# Autodesk Inventor assembly: Podstawa_zlozona+Sruby
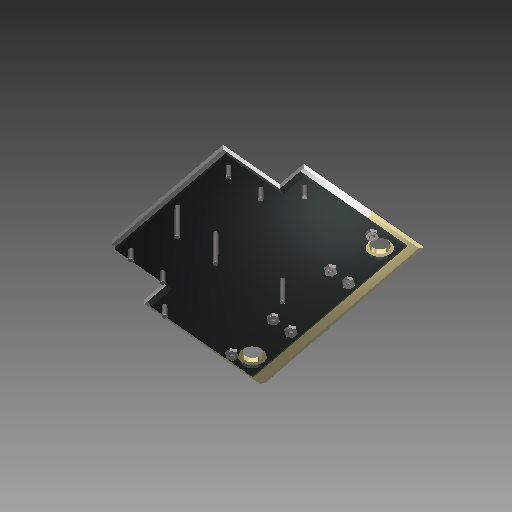
[picture p0: Inventor's stored thumbnail of the model, 512x512]
Saved by Autodesk Inventor 2017 (Build 210142000, 142)
## iProperties
Created: 2016-11-21
Part Number: Podstawa_zlozona+Sruby
Document SubType Name: Assembly
Designer: Shichi
Author: Shichi
## Documents named in this file (7)
- C:\Users\Shichi\Desktop\TooStronk\Podstawy\Podstawa_zlozona+Sruby.iam
- C:\Users\Shichi\Desktop\TooStronk\Podstawy\Podstawa_zlozona.iam
- C:\Users\Shichi\Documents\Inventor\Content Center Files\R2017\en-US\AS 1110\AS 1110 - M2,5 x 12.ipt
- C:\Users\Shichi\Documents\Inventor\Content Center Files\R2017\en-US\AS 1112 (2)\AS 1112 - M2,5  Type 5.ipt
- C:\Users\Shichi\Documents\Inventor\Content Center Files\R2017\en-US\AS 1110\AS 1110 - M2,5 x 8.ipt
- C:\Users\Shichi\Documents\Inventor\Content Center Files\R2017\en-US\AS 1110\AS 1110 - M2,5 x 20.ipt
- C:\Users\Shichi\Documents\Inventor\Content Center Files\R2017\en-US\AS 1110\AS 1110 - M2,5 x 25.ipt
## Components (22 placed, 6 different names)
1. Podstawa_zlozona:1 [sub-assembly] — Insert:1, Insert:2, Insert:4, Insert:5, Insert:6, Insert:7, Insert:10, Insert:11, Insert:12, Insert:13, Insert:14, Insert:15, Insert:16, Insert:17, Insert:18, Insert:19, Insert:20, Insert:21, Insert:22, Insert:23, Insert:24
2. AS 1110 - Metric M2,5 x 12:1 — Insert:4
3. AS 1110 - Metric M2,5 x 8:1 — Insert:11
4. AS 1110 - Metric M2,5 x 12:2 — Insert:2
5. AS 1110 - Metric M2,5 x 12:3 — Insert:5
6. AS 1110 - Metric M2,5 x 12:5 — Insert:1
7. AS 1110 - Metric M2,5 x 12:6 — Insert:6
8. AS 1110 - Metric M2,5 x 8:3 — Insert:15
9. AS 1110 - Metric M2,5 x 8:4 — Insert:14
10. AS 1110 - Metric M2,5 x 8:5 — Insert:13
11. AS 1110 - Metric M2,5 x 8:6 — Insert:12
12. AS 1110 - Metric M2,5 x 8:7 — Insert:10
13. AS 1112 (2) - Metric M2,5  Type 5:3 — Insert:20
14. AS 1112 (2) - Metric M2,5  Type 5:4 — Insert:21
15. AS 1112 (2) - Metric M2,5  Type 5:8 — Insert:17
16. AS 1112 (2) - Metric M2,5  Type 5:9 — Insert:18
17. AS 1112 (2) - Metric M2,5  Type 5:10 — Insert:19
18. AS 1112 (2) - Metric M2,5  Type 5:11 — Insert:16
19. AS 1110 - Metric M2,5 x 12:7 — Insert:7
20. AS 1110 - Metric M2,5 x 20:1 — Insert:22
21. AS 1110 - Metric M2,5 x 25:1 — Insert:24
22. AS 1110 - Metric M2,5 x 25:2 — Insert:23
## Relationships (21: Insert 21)
- Insert:1: Podstawa_zlozona:1 ↔ AS 1110 - Metric M2,5 x 12:5
- Insert:2: Podstawa_zlozona:1 ↔ AS 1110 - Metric M2,5 x 12:2
- Insert:4: Podstawa_zlozona:1 ↔ AS 1110 - Metric M2,5 x 12:1
- Insert:5: Podstawa_zlozona:1 ↔ AS 1110 - Metric M2,5 x 12:3
- Insert:6: Podstawa_zlozona:1 ↔ AS 1110 - Metric M2,5 x 12:6
- Insert:7: Podstawa_zlozona:1 ↔ AS 1110 - Metric M2,5 x 12:7
- Insert:10: Podstawa_zlozona:1 ↔ AS 1110 - Metric M2,5 x 8:7
- Insert:11: Podstawa_zlozona:1 ↔ AS 1110 - Metric M2,5 x 8:1
- Insert:12: Podstawa_zlozona:1 ↔ AS 1110 - Metric M2,5 x 8:6
- Insert:13: Podstawa_zlozona:1 ↔ AS 1110 - Metric M2,5 x 8:5
- Insert:14: Podstawa_zlozona:1 ↔ AS 1110 - Metric M2,5 x 8:4
- Insert:15: Podstawa_zlozona:1 ↔ AS 1110 - Metric M2,5 x 8:3
- Insert:16: Podstawa_zlozona:1 ↔ AS 1112 (2) - Metric M2,5  Type 5:11
- Insert:17: Podstawa_zlozona:1 ↔ AS 1112 (2) - Metric M2,5  Type 5:8
- Insert:18: Podstawa_zlozona:1 ↔ AS 1112 (2) - Metric M2,5  Type 5:9
- Insert:19: Podstawa_zlozona:1 ↔ AS 1112 (2) - Metric M2,5  Type 5:10
- Insert:20: Podstawa_zlozona:1 ↔ AS 1112 (2) - Metric M2,5  Type 5:3
- Insert:21: Podstawa_zlozona:1 ↔ AS 1112 (2) - Metric M2,5  Type 5:4
- Insert:22: Podstawa_zlozona:1 ↔ AS 1110 - Metric M2,5 x 20:1
- Insert:23: Podstawa_zlozona:1 ↔ AS 1110 - Metric M2,5 x 25:2
- Insert:24: Podstawa_zlozona:1 ↔ AS 1110 - Metric M2,5 x 25:1
